# Autodesk Inventor assembly: s-assy-base
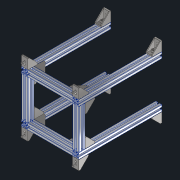
[picture p0: Inventor's stored thumbnail of the model, 180x180]
Saved by Autodesk Inventor 2022 (Build 260153000, 153)
## iProperties
Created: 2021-10-19
Part Number: s-assy-base
Document SubType Name: Assembly
Designer: Yuta Kage
Author: Yuta Kage
## Documents named in this file (7)
- C:\Users\yuta0\Documents\GitHub\catchrobo_hardware\assy-scara\s-assy-base.iam
- C:\Users\yuta0\Documents\GitHub\catchrobo_hardware\assy-scara\NFS5-2020_1.ipt
- C:\Users\yuta0\Documents\GitHub\catchrobo_hardware\assy-scara\NFS5-2020_2.ipt
- C:\Users\yuta0\Documents\GitHub\catchrobo_hardware\assy-shooter\s-assy-blacket.iam
- C:\Users\yuta0\Documents\GitHub\catchrobo_hardware\assy-scara\s-assy-blacket2.iam
- C:\Users\yuta0\Documents\GitHub\catchrobo_hardware\assy-scara\CB5-15.ipt
- C:\Users\yuta0\Documents\GitHub\catchrobo_hardware\assy-scara\NFS5-2020_3.ipt
## Components (28 placed, 6 different names)
1. s-assy-blacket2:3 [sub-assembly] — フラッシュ:28, メイト:25, フラッシュ:31
2. NFS5-2020_1:3 — フラッシュ:2, メイト:1, フラッシュ:3, メイト:6, メイト:11, フラッシュ:19, メイト:17, フラッシュ:28, メイト:21, フラッシュ:29, フラッシュ:30, メイト:25, フラッシュ:31, フラッシュ:33, フラッシュ:34
3. s-assy-blacket:7 [sub-assembly] — フラッシュ:22, メイト:16, メイト:17, フラッシュ:33
4. NFS5-2020_3:1 — メイト:6, メイト:7, メイト:14, フラッシュ:21, フラッシュ:22, メイト:16, フラッシュ:34
5. s-assy-blacket:6 [sub-assembly] — メイト:14, メイト:15, フラッシュ:21
6. NFS5-2020_1:5 — メイト:7, メイト:15, メイト:18, フラッシュ:23, フラッシュ:24, メイト:19, フラッシュ:25, フラッシュ:26, フラッシュ:32
7. s-assy-blacket2:2 [sub-assembly] — メイト:19, フラッシュ:25, フラッシュ:26
8. s-assy-blacket2:1 [sub-assembly] — メイト:18, フラッシュ:23, フラッシュ:24
9. s-assy-blacket2:7 [sub-assembly] — メイト:21, フラッシュ:29, フラッシュ:30
10. s-assy-blacket2:4 [sub-assembly]
11. NFS5-2020_1:6
12. s-assy-blacket:8 [sub-assembly]
13. NFS5-2020_3:2
14. s-assy-blacket:9 [sub-assembly]
15. NFS5-2020_1:7
16. s-assy-blacket2:5 [sub-assembly]
17. s-assy-blacket2:6 [sub-assembly] — メイト:23, メイト:24
18. s-assy-blacket2:8 [sub-assembly]
19. NFS5-2020_2:1 — フラッシュ:2, メイト:1, フラッシュ:3, メイト:12, メイト:13
20. s-assy-blacket:3 [sub-assembly] — メイト:12
21. s-assy-blacket:2 [sub-assembly] — メイト:11, メイト:13, フラッシュ:19
22. NFS5-2020_2:4 — フラッシュ:32
23. s-assy-blacket:10 [sub-assembly]
24. s-assy-blacket:11 [sub-assembly]
25. CB5-15:1 — メイト:23, メイト:24
26. CB5-15:2
27. CB5-15:3
28. CB5-15:4
## Component patterns: (2 elements, first: s-assy-blacket2:3 + NFS5-2020_1:3 + s-assy-blacket:7 + NFS5-2020_3:1 + s-assy-blacket:6 + NFS5-2020_1:5 + s-assy-blacket2:2 + s-assy-blacket2:1 + s-assy-blacket2:7), (2 elements, first: NFS5-2020_2:1 + s-assy-blacket:3 + s-assy-blacket:2), (4 elements, first: CB5-15:1)
## Relationships (32: Flush 16, Mate 16)
- フラッシュ:2 [Flush]: NFS5-2020_1:3 ↔ NFS5-2020_2:1
- メイト:1 [Mate]: NFS5-2020_1:3 ↔ NFS5-2020_2:1
- フラッシュ:3 [Flush]: NFS5-2020_1:3 ↔ NFS5-2020_2:1
- メイト:6 [Mate]: NFS5-2020_1:3 ↔ NFS5-2020_3:1
- メイト:7 [Mate]: NFS5-2020_3:1 ↔ NFS5-2020_1:5
- メイト:11 [Mate]: NFS5-2020_1:3 ↔ s-assy-blacket:2
- メイト:12 [Mate]: NFS5-2020_2:1 ↔ s-assy-blacket:3
- メイト:13 [Mate]: NFS5-2020_2:1 ↔ s-assy-blacket:2
- フラッシュ:19 [Flush]: NFS5-2020_1:3 ↔ s-assy-blacket:2
- メイト:14 [Mate]: NFS5-2020_3:1 ↔ s-assy-blacket:6
- メイト:15 [Mate]: s-assy-blacket:6 ↔ NFS5-2020_1:5
- フラッシュ:21 [Flush]: NFS5-2020_3:1 ↔ s-assy-blacket:6
- フラッシュ:22 [Flush]: s-assy-blacket:7 ↔ NFS5-2020_3:1
- メイト:16 [Mate]: s-assy-blacket:7 ↔ NFS5-2020_3:1
- メイト:17 [Mate]: NFS5-2020_1:3 ↔ s-assy-blacket:7
- メイト:18 [Mate]: NFS5-2020_1:5 ↔ s-assy-blacket2:1
- フラッシュ:23 [Flush]: NFS5-2020_1:5 ↔ s-assy-blacket2:1
- フラッシュ:24 [Flush]: NFS5-2020_1:5 ↔ s-assy-blacket2:1
- メイト:19 [Mate]: NFS5-2020_1:5 ↔ s-assy-blacket2:2
- フラッシュ:25 [Flush]: NFS5-2020_1:5 ↔ s-assy-blacket2:2
- フラッシュ:26 [Flush]: NFS5-2020_1:5 ↔ s-assy-blacket2:2
- フラッシュ:28 [Flush]: s-assy-blacket2:3 ↔ NFS5-2020_1:3
- メイト:21 [Mate]: NFS5-2020_1:3 ↔ s-assy-blacket2:7
- フラッシュ:29 [Flush]: NFS5-2020_1:3 ↔ s-assy-blacket2:7
- フラッシュ:30 [Flush]: NFS5-2020_1:3 ↔ s-assy-blacket2:7
- メイト:23 [Mate]: s-assy-blacket2:6 ↔ CB5-15:1
- メイト:24 [Mate]: s-assy-blacket2:6 ↔ CB5-15:1
- メイト:25 [Mate]: s-assy-blacket2:3 ↔ NFS5-2020_1:3
- フラッシュ:31 [Flush]: s-assy-blacket2:3 ↔ NFS5-2020_1:3
- フラッシュ:32 [Flush]: NFS5-2020_1:5 ↔ NFS5-2020_2:4
- フラッシュ:33 [Flush]: NFS5-2020_1:3 ↔ s-assy-blacket:7
- フラッシュ:34 [Flush]: NFS5-2020_1:3 ↔ NFS5-2020_3:1
